# Autodesk Inventor assembly: Overall_Shooting_Mechanism2
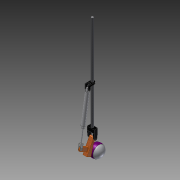
[picture p0: Inventor's stored thumbnail of the model, 180x180]
Saved by Autodesk Inventor 2015 (Build 190159000, 159)
## iProperties
Created: 2017-02-21
Part Number: Overall_Shooting_Mechanism2
Document SubType Name: Assembly
Designer: Guy
Author: Guy
## Documents named in this file (9)
- C:\Users\Guy\Documents\Fourth Year\Capstone\git\Capstone-Project\doc\CAD\SM2\Overall_Shooting_Mechanism2.iam
- C:\Users\Guy\Documents\Fourth Year\Capstone\git\Capstone-Project\doc\CAD\SM2\Swinging_connection.ipt
- C:\Users\Guy\Documents\Fourth Year\Capstone\git\Capstone-Project\doc\CAD\SM2\hinge_for_swing.ipt
- C:\Users\Guy\Documents\Fourth Year\Capstone\git\Capstone-Project\doc\CAD\ShootingMechanism\MountBar.ipt
- C:\Users\Guy\Documents\Fourth Year\Capstone\git\Capstone-Project\doc\CAD\SM2\Piston_Holder.ipt
- C:\Users\Guy\Documents\Fourth Year\Capstone\git\Capstone-Project\doc\CAD\SM2\Small_piston.ipt
- C:\Users\Guy\Documents\Fourth Year\Capstone\git\Capstone-Project\doc\CAD\SM2\piston_rod_connector.ipt
- C:\Users\Guy\Documents\Fourth Year\Capstone\git\Capstone-Project\doc\CAD\SM2\piston_internal_rod.ipt
- C:\Users\Guy\Documents\Fourth Year\Capstone\git\Capstone-Project\doc\CAD\LowLevel_Rev2\Pool_Ball_Stripe.ipt
## Components (8 placed, 8 different names)
1. hinge_for_swing:2 — Mate:3, Angle:1, Flush:4, Mate:29, Mate:32, Mate:34
2. MountBar:1 — Mate:3, Angle:1, Flush:4, Mate:15, Mate:20, Angle:2
3. Pool_Ball_Stripe:1 — Mate:15
4. Piston_Holder:1 — Mate:20, Mate:26, Mate:29, Mate:30, Angle:2
5. piston_internal_rod:1 — Mate:21, Mate:22, Flush:5
6. piston_rod_connector:1 — Mate:21, Flush:5, Mate:31, Mate:33
7. Small_piston:1 — Mate:22, Mate:26, Mate:30, Mate:31
8. Swinging_connection:1 — Mate:32, Mate:33, Mate:34
## Relationships (16: Mate 12, Angle 2, Flush 2)
- Mate:3: hinge_for_swing:2 ↔ MountBar:1
- Angle:1 (0 deg): hinge_for_swing:2 ↔ MountBar:1
- Flush:4 (-5 mm): hinge_for_swing:2 ↔ MountBar:1
- Mate:15: MountBar:1 ↔ Pool_Ball_Stripe:1
- Mate:20: MountBar:1 ↔ Piston_Holder:1
- Mate:21: piston_internal_rod:1 ↔ piston_rod_connector:1
- Mate:22: piston_internal_rod:1 ↔ Small_piston:1
- Flush:5: piston_internal_rod:1 ↔ piston_rod_connector:1
- Mate:26: Piston_Holder:1 ↔ Small_piston:1
- Mate:29 (170 mm): hinge_for_swing:2 ↔ Piston_Holder:1
- Mate:30 (1 mm): Piston_Holder:1 ↔ Small_piston:1
- Angle:2 (-90 deg): MountBar:1 ↔ Piston_Holder:1
- Mate:31 (56.34 mm): piston_rod_connector:1 ↔ Small_piston:1
- Mate:32: hinge_for_swing:2 ↔ Swinging_connection:1
- Mate:33: piston_rod_connector:1 ↔ Swinging_connection:1
- Mate:34 (0.5 mm): hinge_for_swing:2 ↔ Swinging_connection:1
